# Autodesk Inventor assembly: Vacubot v1
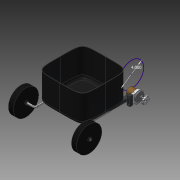
[picture p0: Inventor's stored thumbnail of the model, 180x180]
Saved by Autodesk Inventor 2014 SP1 (Build 180222100, 222)
## iProperties
Created: 2013-12-26
Part Number: Vacubot v1
Document SubType Name: Assembly
Designer: tom
Author: tom
## Documents named in this file (11)
- C:\Users\tom\Documents\GitHub\Vacubot\Inventor\Vacubot v1.iam
- C:\Users\tom\Documents\GitHub\Vacubot\Inventor\Base.ipt
- C:\Users\tom\Documents\GitHub\Vacubot\Inventor\Base Plate.ipt
- C:\Users\tom\Documents\GitHub\Vacubot\Inventor\Motor Mount.ipt
- C:\Users\tom\Documents\GitHub\Vacubot\Inventor\Wheel Original.iam
- C:\Users\tom\Documents\GitHub\Vacubot\Inventor\Wheel Original_MIR.iam
- C:\Users\tom\Documents\GitHub\Vacubot\Inventor\Drive Motor.ipt
- C:\Users\tom\Documents\GitHub\Vacubot\Inventor\Clamping Hub.ipt
- C:\Users\tom\Documents\GitHub\Vacubot\Inventor\Motor Mount_MIR1.ipt
- C:\Users\tom\Documents\GitHub\Vacubot\Inventor\Drive Motor_MIR.ipt
- C:\Users\tom\Documents\GitHub\Vacubot\Inventor\Wheel.ipt
## Components (10 placed, 10 different names)
1. Chassis — Mate:9, Mate:10, Mate:11, Mate:14, Mate:15
2. Base Plate:1
3. Motor Mount:1 — Mate:8, Flush:1, Mate:9, Mate:10, Mate:11
4. Wheel Original:1 [sub-assembly]
5. Wheel Original_MIR:1 [sub-assembly]
6. Drive Motor:1 — Mate:8, Flush:1, Mate:13, Mate:16, Mate:17
7. Clamping Hub:1 — Mate:16, Mate:17
8. Motor Mount_MIR1:1 — Flush:2, Mate:12, Mate:14, Mate:15
9. Drive Motor_MIR:1 — Flush:2, Mate:12, Mate:13
10. Wheel:1
## Relationships (15: Mate 12, Flush 2, Tangent 1)
- [Mate] (-6.35 mm): Wheel Original:1
- [Tangent]: Chassis ↔ Wheel Original:1
- [Mate] (-6.35 mm): Wheel Original:1
- Mate:8: Motor Mount:1 ↔ Drive Motor:1
- Flush:1 (-5 mm): Motor Mount:1 ↔ Drive Motor:1
- Mate:9: Chassis ↔ Motor Mount:1
- Mate:10: Chassis ↔ Motor Mount:1
- Mate:11: Chassis ↔ Motor Mount:1
- Flush:2 (-5 mm): Motor Mount_MIR1:1 ↔ Drive Motor_MIR:1
- Mate:12: Motor Mount_MIR1:1 ↔ Drive Motor_MIR:1
- Mate:13: Drive Motor:1 ↔ Drive Motor_MIR:1
- Mate:14: Chassis ↔ Motor Mount_MIR1:1
- Mate:15: Chassis ↔ Motor Mount_MIR1:1
- Mate:16: Drive Motor:1 ↔ Clamping Hub:1
- Mate:17: Drive Motor:1 ↔ Clamping Hub:1
